# Autodesk Inventor assembly: main
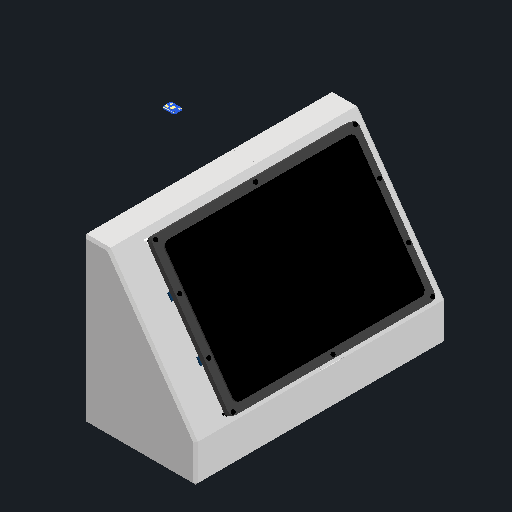
[picture p0: Inventor's stored thumbnail of the model, 512x512]
Saved by Autodesk Inventor 2026.2 (Build 302298000, 298)
## iProperties
Created: 2025-12-22
Part Number: main
Document SubType Name: Assembly
Designer: test
wood_thickness: 10.000 mm
Author: test
## Documents named in this file (9)
- D:\Projects\spl-monitor\simple-concert-monitor_Mechanical\main.iam
- D:\Projects\spl-monitor\simple-concert-monitor_Mechanical\screen\screen.iam
- D:\Projects\spl-monitor\simple-concert-monitor_Mechanical\external\raspberry-pi-4-model-b-1.snapshot.3\Raspberry Pi 4 Model B\Raspberry Pi 4 Model B\Raspberry Pi 4 Model B.iam
- D:\Projects\spl-monitor\simple-concert-monitor_Mechanical\external\adafruit-i2s-pi-mic-breakout-sph0645-1.snapshot.1\Pi Mic breakout SPH0645\Pi Mic breakout SPH0645\Pi Mic breakout SPH0645.ipt
- D:\Projects\spl-monitor\simple-concert-monitor_Mechanical\external\on-off-kcd4-220v-6a-1.snapshot.1\ON-OFF KCD4 220V 6A\ON-OFF KCD4 220V 6A\ON-OFF KCD4 220V 6A.iam
- D:\Projects\spl-monitor\simple-concert-monitor_Mechanical\external\ss-7b-as-207-ac-1-1.snapshot.3\SS-7B Socket\Plug SS-7B\Plug SS-7B\Plug SS-7B.ipt
- D:\Projects\spl-monitor\simple-concert-monitor_Mechanical\case3.ipt
- D:\Projects\spl-monitor\simple-concert-monitor_Mechanical\case4.ipt
- D:\Projects\spl-monitor\simple-concert-monitor_Mechanical\case5.ipt
## Components (8 placed, 8 different names)
1. screen:1 [sub-assembly] — Mate:1, Mate:2, Mate:3, Mate:4
2. Raspberry Pi 4 Model B:1 [sub-assembly] — Angle:1
3. Pi Mic breakout SPH0645:1
4. ON-OFF KCD4 220V 6A:1 [sub-assembly] — Mate:6, Mate:7, Mate:8
5. Plug SS-7B:1 — Mate:5, Mate:9, Mate:10
6. case3:1 — Mate:1, Mate:2, Mate:3, Flush:1, Mate:12, Flush:2, Angle:1
7. case4:1 — Flush:1, Mate:4, Mate:5, Mate:6, Mate:7, Mate:8, Mate:9, Mate:10, Mate:11
8. case5:1 — Mate:11, Mate:12, Flush:2
## Relationships (15: Mate 12, Flush 2, Angle 1)
- Mate:1: screen:1 ↔ case3:1
- Mate:2: screen:1 ↔ case3:1
- Mate:3: screen:1 ↔ case3:1
- Flush:1: case3:1 ↔ case4:1
- Mate:4: screen:1 ↔ case4:1
- Mate:5: Plug SS-7B:1 ↔ case4:1
- Mate:6: ON-OFF KCD4 220V 6A:1 ↔ case4:1
- Mate:7: ON-OFF KCD4 220V 6A:1 ↔ case4:1
- Mate:8: ON-OFF KCD4 220V 6A:1 ↔ case4:1
- Mate:9: Plug SS-7B:1 ↔ case4:1
- Mate:10: Plug SS-7B:1 ↔ case4:1
- Mate:11: case4:1 ↔ case5:1
- Mate:12: case3:1 ↔ case5:1
- Flush:2: case3:1 ↔ case5:1
- Angle:1 (0 deg): Raspberry Pi 4 Model B:1 ↔ case3:1
